# Autodesk Inventor assembly: 関節3
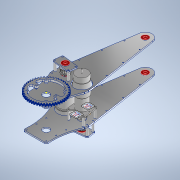
[picture p0: Inventor's stored thumbnail of the model, 180x180]
Saved by Autodesk Inventor 2021 (Build 250183000, 183)
## iProperties
Created: 2022-02-02
Part Number: 関節3
Document SubType Name: Assembly
Designer: hirohumi
Author: hirohumi
## Documents named in this file (19)
- C:\Users\hirohumi\OneDrive\ドキュメント\ロボ研\2022NHKロボコン\R2_version1\3軸アームver2\関節3.iam
- C:\Users\hirohumi\OneDrive\ドキュメント\ロボ研\2022NHKロボコン\R2_version1\3軸アームver2\関節3_側板1.ipt
- C:\Users\hirohumi\OneDrive\ドキュメント\ロボ研\2022NHKロボコン\R2_version1\3軸アーム\軸6-25.ipt
- C:\Users\hirohumi\OneDrive\ドキュメント\ロボ研\2022NHKロボコン\R2_version1\3軸アーム\関節3_555側_モータマウント.ipt
- C:\Users\hirohumi\OneDrive\ドキュメント\ロボ研\2022NHKロボコン\R2_version1\RS-555-71.ipt
- C:\Users\hirohumi\OneDrive\ドキュメント\ロボ研\2022NHKロボコン\R2_version1\3軸アーム\カップリング_軸6mm.ipt
- C:\Users\hirohumi\OneDrive\ドキュメント\ロボ研\2022NHKロボコン\R2_version1\3軸アーム\カップリング_軸8mm_2.5mm.ipt
- C:\Users\hirohumi\OneDrive\ドキュメント\ロボ研\2022NHKロボコン\R2_version1\3軸アーム\軸8-30.ipt
- C:\Users\hirohumi\OneDrive\ドキュメント\ロボ研\2022NHKロボコン\R2_version1\3軸アーム\プーリ_歯数15.ipt
- C:\Users\hirohumi\OneDrive\ドキュメント\ロボ研\2022NHKロボコン\R2_version1\3軸アーム\プーリ_歯数15_2.5mm.ipt
- C:\Users\hirohumi\OneDrive\ドキュメント\ロボ研\2022NHKロボコン\R2_version1\3軸アーム\カップリング_軸8mm.ipt
- C:\Users\hirohumi\OneDrive\ドキュメント\ロボ研\2022NHKロボコン\R2_version1\3軸アーム\AMT102Normal\CUI_DEVICES_AMT102-0048-N8000-S.iam
- C:\Users\hirohumi\OneDrive\ドキュメント\ロボ研\2022NHKロボコン\R2_version1\3軸アーム\関節3_775側_モータマウント.ipt
- C:\Users\hirohumi\OneDrive\ドキュメント\ロボ研\2022NHKロボコン\R2_version1\RS-775GM104 v1.ipt
- C:\Users\hirohumi\OneDrive\ドキュメント\ロボ研\2022NHKロボコン\R2_version1\3軸アーム\エンコーダマウント.ipt
- C:\Users\hirohumi\OneDrive\ドキュメント\ロボ研\2022NHKロボコン\R2_version1\3軸アーム\ベアリングフランジ付き.ipt
- C:\Users\hirohumi\OneDrive\ドキュメント\ロボ研\2022NHKロボコン\R2_version1\3軸アーム\軸6-5.ipt
- C:\Users\hirohumi\OneDrive\ドキュメント\ロボ研\2022NHKロボコン\R2_version1\3軸アーム\ギア_歯数50.ipt
- C:\Users\hirohumi\OneDrive\ドキュメント\ロボ研\2022NHKロボコン\R2_version1\3軸アームver2\関節3_プーリ側板.ipt
## Components (48 placed, 18 different names)
1. 関節3_側板1:1 — 挿入:19, 挿入:20, 挿入:21, 挿入:22, メイト:4, 挿入:46, 挿入:47, 挿入:48, 挿入:49, 挿入:50, 挿入:51
2. 関節3_側板1:2 — 挿入:23, 挿入:42, 挿入:43, メイト:4, 挿入:52, 挿入:53, 挿入:54, 挿入:55
3. 軸6-25:1 — 挿入:18, 挿入:19
4. 軸6-25:2
5. 軸6-25:3
6. 軸6-25:4 — 挿入:17, 挿入:20
7. 関節3_775側_モータマウント:1 — 挿入:17, 挿入:18
8. RS-775GM104 v1:1
9. カップリング_軸8mm:1
10. カップリング_軸8mm_2.5mm:1
11. 軸8-30:1
12. プーリ_歯数15:1
13. プーリ_歯数15_2.5mm:1
14. カップリング_軸8mm:2
15. CUI_DEVICES_AMT102-0048-N8000-S:1 [sub-assembly]
16. エンコーダマウント:1
17. ベアリングフランジ付き:1 — 挿入:21
18. ベアリングフランジ付き:2 — 挿入:23, メイト:3
19. ベアリングフランジ付き:3 — 挿入:22, メイト:3
20. 軸6-25:5
21. 軸6-25:6 — 挿入:41
22. 軸6-25:7 — 挿入:43
23. 軸6-25:8 — 挿入:40, 挿入:42
24. 関節3_555側_モータマウント:1 — 挿入:40, 挿入:41
25. RS-555-71:1
26. カップリング_軸6mm:1
27. カップリング_軸8mm_2.5mm:2
28. 軸8-30:2
29. プーリ_歯数15:2
30. プーリ_歯数15_2.5mm:2
31. カップリング_軸8mm:3
32. CUI_DEVICES_AMT102-0048-N8000-S:2 [sub-assembly]
33. エンコーダマウント:2
34. 軸6-5:1 — 挿入:46
35. 軸6-5:2 — 挿入:47
36. ギア_歯数50:1
37. 軸6-25:9 — 挿入:48, 挿入:59
38. 軸6-25:10 — 挿入:49
39. 軸6-25:11 — 挿入:50, 挿入:58
40. 軸6-25:12 — 挿入:51
41. 軸6-25:13 — 挿入:52, 挿入:56
42. 軸6-25:14 — 挿入:53, 挿入:57
43. 軸6-25:15 — 挿入:54
44. 軸6-25:16 — 挿入:55
45. 関節3_プーリ側板:1 — 挿入:56, 挿入:57, 挿入:61
46. 関節3_プーリ側板:2 — 挿入:58, 挿入:59, 挿入:60
47. ベアリングフランジ付き:4 — 挿入:60
48. ベアリングフランジ付き:5 — 挿入:61
## Relationships (65: Insert 61, Mate 4)
- [Insert]: 軸6-25:2 ↔ 関節3_775側_モータマウント:1
- [Insert]: 軸6-25:3 ↔ 関節3_775側_モータマウント:1
- [Insert]: 関節3_775側_モータマウント:1 ↔ RS-775GM104 v1:1
- [Insert]: 関節3_775側_モータマウント:1 ↔ RS-775GM104 v1:1
- [Insert]: カップリング_軸8mm:1 ↔ カップリング_軸8mm_2.5mm:1
- [Insert]: カップリング_軸8mm:1 ↔ カップリング_軸8mm_2.5mm:1
- [Insert]: RS-775GM104 v1:1 ↔ カップリング_軸8mm_2.5mm:1
- [Insert]: カップリング_軸8mm_2.5mm:1 ↔ 軸8-30:1
- [Insert]: プーリ_歯数15:1 ↔ プーリ_歯数15_2.5mm:1
- [Insert]: プーリ_歯数15:1 ↔ プーリ_歯数15_2.5mm:1
- [Insert]: プーリ_歯数15:1 ↔ カップリング_軸8mm:2
- [Insert]: プーリ_歯数15:1 ↔ カップリング_軸8mm:2
- [Mate]: 軸8-30:1 ↔ カップリング_軸8mm:2
- [Insert]: CUI_DEVICES_AMT102-0048-N8000-S:1 ↔ エンコーダマウント:1
- [Insert]: CUI_DEVICES_AMT102-0048-N8000-S:1 ↔ エンコーダマウント:1
- [Insert]: 関節3_775側_モータマウント:1 ↔ エンコーダマウント:1
- [Insert]: 関節3_775側_モータマウント:1 ↔ エンコーダマウント:1
- 挿入:17 [Insert]: 軸6-25:4 ↔ 関節3_775側_モータマウント:1
- 挿入:18 [Insert]: 軸6-25:1 ↔ 関節3_775側_モータマウント:1
- 挿入:19 [Insert]: 関節3_側板1:1 ↔ 軸6-25:1
- 挿入:20 [Insert]: 関節3_側板1:1 ↔ 軸6-25:4
- 挿入:21 [Insert]: 関節3_側板1:1 ↔ ベアリングフランジ付き:1
- 挿入:22 [Insert]: 関節3_側板1:1 ↔ ベアリングフランジ付き:3
- 挿入:23 [Insert]: 関節3_側板1:2 ↔ ベアリングフランジ付き:2
- [Insert]: 軸6-25:5 ↔ 関節3_555側_モータマウント:1
- [Insert]: 軸6-25:7 ↔ 関節3_555側_モータマウント:1
- [Insert]: 関節3_555側_モータマウント:1 ↔ RS-555-71:1
- [Insert]: 関節3_555側_モータマウント:1 ↔ RS-555-71:1
- [Insert]: カップリング_軸6mm:1 ↔ カップリング_軸8mm_2.5mm:2
- [Insert]: カップリング_軸6mm:1 ↔ カップリング_軸8mm_2.5mm:2
- [Insert]: RS-555-71:1 ↔ カップリング_軸6mm:1
- [Insert]: カップリング_軸6mm:1 ↔ 軸8-30:2
- [Insert]: プーリ_歯数15:2 ↔ プーリ_歯数15_2.5mm:2
- [Insert]: プーリ_歯数15:2 ↔ プーリ_歯数15_2.5mm:2
- [Insert]: プーリ_歯数15:2 ↔ カップリング_軸8mm:3
- [Insert]: プーリ_歯数15:2 ↔ カップリング_軸8mm:3
- [Mate]: 軸8-30:2 ↔ カップリング_軸8mm:3
- [Insert]: CUI_DEVICES_AMT102-0048-N8000-S:2 ↔ エンコーダマウント:2
- [Insert]: CUI_DEVICES_AMT102-0048-N8000-S:2 ↔ エンコーダマウント:2
- [Insert]: 関節3_555側_モータマウント:1 ↔ エンコーダマウント:2
- [Insert]: 関節3_555側_モータマウント:1 ↔ エンコーダマウント:2
- 挿入:40 [Insert]: 軸6-25:8 ↔ 関節3_555側_モータマウント:1
- 挿入:41 [Insert]: 軸6-25:6 ↔ 関節3_555側_モータマウント:1
- 挿入:42 [Insert]: 関節3_側板1:2 ↔ 軸6-25:8
- 挿入:43 [Insert]: 関節3_側板1:2 ↔ 軸6-25:7
- メイト:3 [Mate]: ベアリングフランジ付き:2 ↔ ベアリングフランジ付き:3
- メイト:4 [Mate]: 関節3_側板1:1 ↔ 関節3_側板1:2
- [Insert]: 軸6-5:1 ↔ ギア_歯数50:1
- [Insert]: 軸6-5:2 ↔ ギア_歯数50:1
- 挿入:46 [Insert]: 関節3_側板1:1 ↔ 軸6-5:1
- 挿入:47 [Insert]: 関節3_側板1:1 ↔ 軸6-5:2
- 挿入:48 [Insert]: 関節3_側板1:1 ↔ 軸6-25:9
- 挿入:49 [Insert]: 関節3_側板1:1 ↔ 軸6-25:10
- 挿入:50 [Insert]: 関節3_側板1:1 ↔ 軸6-25:11
- 挿入:51 [Insert]: 関節3_側板1:1 ↔ 軸6-25:12
- 挿入:52 [Insert]: 関節3_側板1:2 ↔ 軸6-25:13
- 挿入:53 [Insert]: 関節3_側板1:2 ↔ 軸6-25:14
- 挿入:54 [Insert]: 関節3_側板1:2 ↔ 軸6-25:15
- 挿入:55 [Insert]: 関節3_側板1:2 ↔ 軸6-25:16
- 挿入:56 [Insert]: 軸6-25:13 ↔ 関節3_プーリ側板:1
- 挿入:57 [Insert]: 軸6-25:14 ↔ 関節3_プーリ側板:1
- 挿入:58 [Insert]: 軸6-25:11 ↔ 関節3_プーリ側板:2
- 挿入:59 [Insert]: 軸6-25:9 ↔ 関節3_プーリ側板:2
- 挿入:60 [Insert]: 関節3_プーリ側板:2 ↔ ベアリングフランジ付き:4
- 挿入:61 [Insert]: 関節3_プーリ側板:1 ↔ ベアリングフランジ付き:5
## Named parameters: d57_d55 = 0 mm, d58_d56 = 0 mm, d59_d53 = 0 mm, d60_d54 = 0 mm, d59_d45 = 0 mm, d60_d46 = 0 mm, d62_d47 = 0 mm, d63_d48 = 0 mm, d64_d49 = 0 mm, d65_d51 = 0 mm
